# Autodesk Inventor assembly: final linear and linkage2
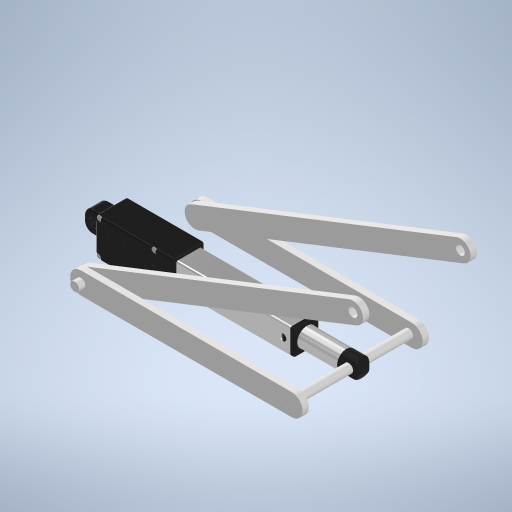
[picture p0: Inventor's stored thumbnail of the model, 512x512]
Saved by Autodesk Inventor 2024.1 (Build 281209000, 209)
## iProperties
Created: 2024-01-24
Part Number: final linear and linkage2
Document SubType Name: Assembly
Designer: udayk
Author: udayk
## Documents named in this file (6)
- C:\Users\udayk\OneDrive\Desktop\Year 1\Engineer IP13\Project 3\My modelling\final linear and linkage2.iam
- C:\Users\udayk\OneDrive\Desktop\Year 1\Engineer IP13\Project 3\Assembly rn\connector linkage_CPY.ipt
- C:\Users\udayk\OneDrive\Desktop\Year 1\Engineer IP13\Project 3\Assembly rn\connector linkage.ipt
- C:\Users\udayk\OneDrive\Desktop\Year 1\Engineer IP13\Project 3\Assembly rn\linkage.ipt
- C:\Users\udayk\OneDrive\Desktop\Year 1\Engineer IP13\Project 3\Assembly rn\inserted rod_CPY.ipt
- C:\Users\udayk\OneDrive\Desktop\Year 1\Engineer IP13\Project 3\Thurs-08 Modelling\2. Hopper Assembly\2. Hopper Assembly\Linear Actuator_CPY.iam
## Components (6 placed, 5 different names)
1. connector linkage_CPYmover:1 — Mate:2, Angle:2, Angle:4, Flush:2, Mate:5, Mate:6, Mate:9
2. linkage:1 — Angle:4, Mate:5, Mate:6, Angle:9
3. linkage:2 — Angle:3, Mate:4, Mate:7, Angle:8
4. connector linkage:1 — Mate:3, Angle:1, Angle:3, Flush:1, Mate:4, Mate:7, Mate:8
5. inserted rod_CPYmover:1 — Mate:1, Mate:2, Mate:3, Flush:1, Flush:2, Angle:5, Angle:6, Angle:7, Flush:3
6. Linear Actuator_CPYmover:1 [sub-assembly] — Mate:1, Angle:1, Angle:2, Angle:5, Angle:6, Angle:7, Flush:3, Mate:8, Mate:9, Angle:8, Angle:9
## Relationships (21: Mate 9, Angle 9, Flush 3)
- Mate:1: inserted rod_CPYmover:1 ↔ Linear Actuator_CPYmover:1
- Mate:2: connector linkage_CPYmover:1 ↔ inserted rod_CPYmover:1
- Mate:3: connector linkage:1 ↔ inserted rod_CPYmover:1
- Angle:1 (0 deg): connector linkage:1 ↔ Linear Actuator_CPYmover:1
- Angle:2 (0 deg): connector linkage_CPYmover:1 ↔ Linear Actuator_CPYmover:1
- Angle:3 (0 deg): linkage:2 ↔ connector linkage:1
- Angle:4 (0 deg): connector linkage_CPYmover:1 ↔ linkage:1
- Flush:1: connector linkage:1 ↔ inserted rod_CPYmover:1
- Flush:2: connector linkage_CPYmover:1 ↔ inserted rod_CPYmover:1
- Angle:5 (0 deg): inserted rod_CPYmover:1 ↔ Linear Actuator_CPYmover:1
- Angle:6 (0 deg): inserted rod_CPYmover:1 ↔ Linear Actuator_CPYmover:1
- Angle:7 (0 deg): inserted rod_CPYmover:1 ↔ Linear Actuator_CPYmover:1
- Flush:3 (-28.5 mm): inserted rod_CPYmover:1 ↔ Linear Actuator_CPYmover:1
- Mate:4: linkage:2 ↔ connector linkage:1
- Mate:5: connector linkage_CPYmover:1 ↔ linkage:1
- Mate:6: connector linkage_CPYmover:1 ↔ linkage:1
- Mate:7: linkage:2 ↔ connector linkage:1
- Mate:8: connector linkage:1 ↔ Linear Actuator_CPYmover:1
- Mate:9: connector linkage_CPYmover:1 ↔ Linear Actuator_CPYmover:1
- Angle:8 (0 deg): linkage:2 ↔ Linear Actuator_CPYmover:1
- Angle:9 (0 deg): linkage:1 ↔ Linear Actuator_CPYmover:1
